# Autodesk Inventor assembly: FrontOdomPod
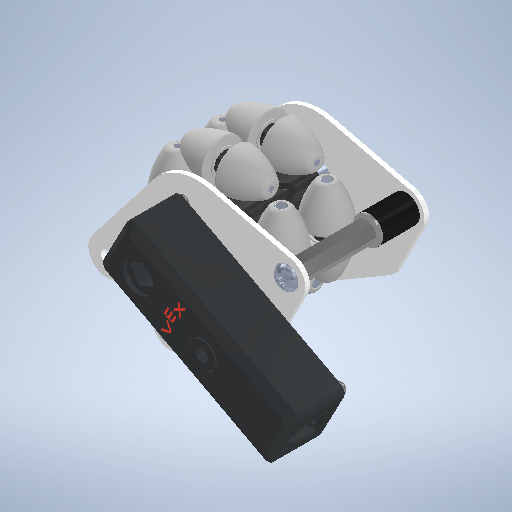
[picture p0: Inventor's stored thumbnail of the model, 512x512]
Saved by Autodesk Inventor 2025.2 (Build 292293000, 293)
## iProperties
Created: 2025-03-23
Part Number: FrontOdomPod
Document SubType Name: Assembly
Designer: roejo
Author: roejo
## Documents named in this file (18)
- C:\1629X-7700R-Worlds-Bot\Bot 1\FrontOdomPod.iam
- C:\1629X-7700R-Worlds-Bot\Bot 1\Plastic\Odom\Front Horizontal Odom Pod nonRot Side.ipt
- C:\1629X-7700R-Worlds-Bot\Bot 1\Plastic\Odom\Front Horizontal Odom Pod Rot Side.ipt
- C:\1629X-7700R-Worlds-Bot\VEX-CAD-Inventor-1.4.2\Motion\Spacers\Washer Steel\SWasher .375 OD x .031250.ipt
- C:\1629X-7700R-Worlds-Bot\VEX-CAD-Inventor-1.4.2\Motion\Spacers\Washer Steel.ipt
- C:\1629X-7700R-Worlds-Bot\VEX-CAD-Inventor-1.4.2\Structure\Standoff\Standoff 1.00.ipt
- C:\1629X-7700R-Worlds-Bot\VEX-CAD-Inventor-1.4.2\Structure\Standoff.ipt
- C:\1629X-7700R-Worlds-Bot\VEX-CAD-Inventor-1.4.2\Motion\Spacers\Spacer Nylon .375 OD\NSpacer .375 OD x .500.ipt
- C:\1629X-7700R-Worlds-Bot\VEX-CAD-Inventor-1.4.2\Motion\Spacers\Spacer Nylon .375 OD.ipt
- C:\1629X-7700R-Worlds-Bot\VEX-CAD-Inventor-1.4.2\Electronics\Sensors\V5 Rotation Sensor.ipt
- C:\1629X-7700R-Worlds-Bot\VEX-CAD-Inventor-1.4.2\Motion\Wheels\Omni Wheel\2 Omni AS, No Insert.ipt
- C:\1629X-7700R-Worlds-Bot\VEX-CAD-Inventor-1.4.2\Motion\Shaft LS\Shaft Collar Metal\Shaft Collar No Screw.iam
- C:\1629X-7700R-Worlds-Bot\VEX-CAD-Inventor-1.4.2\Motion\Shaft LS\Shaft Collar Metal.iam
- C:\1629X-7700R-Worlds-Bot\VEX-CAD-Inventor-1.4.2\Motion\Spacers\Washer Teflon\TWasher .375 OD x .04000.ipt
- C:\1629X-7700R-Worlds-Bot\VEX-CAD-Inventor-1.4.2\Motion\Spacers\Washer Teflon.ipt
- C:\1629X-7700R-Worlds-Bot\VEX-CAD-Inventor-1.4.2\Structure\Hardware\Screw Steel - Star.ipt
- C:\1629X-7700R-Worlds-Bot\VEX-CAD-Inventor-1.4.2\Structure\Hardware\Screw Steel - Star\SScrew Star Smooth .375.ipt
- C:\1629X-7700R-Worlds-Bot\VEX-CAD-Inventor-1.4.2\Structure\Hardware\Screw Steel - Star\SScrew Star Smooth .875.ipt
## Components (19 placed, 11 different names)
1. Front Horizontal Odom Pod nonRot Side:1 — Insert:5, Insert:11, Insert:12, Insert:17, Insert:18
2. Front Horizontal Odom Pod Rot Side:1 — Insert:1, Insert:9, Insert:10, Insert:19, Insert:20
3. SWasher .375 OD x .031250:1 — Insert:3, Insert:4
4. SWasher .375 OD x .031250:2 — Insert:1, Insert:2
5. Standoff 1.00:1 — Insert:2, Insert:3
6. NSpacer .375 OD x .500:1 — Insert:4, Insert:5
7. SWasher .375 OD x .031250:3
8. SWasher .375 OD x .031250:4 — Insert:9
9. Standoff 1.00:2
10. NSpacer .375 OD x .500:2 — Insert:11
11. V5 Rotation Sensor:1 — Insert:10
12. 2 Omni AS, No Insert:1 — Insert:13, Insert:14
13. Shaft Collar No Screw:1 [sub-assembly] — Insert:12, Insert:13
14. 2 Omni AS, No Insert:2 — Insert:14, Insert:15
15. TWasher .375 OD x .04000:1 — Insert:15
16. SScrew Star Smooth .375:3 — Insert:19
17. SScrew Star Smooth .375:4 — Insert:20
18. SScrew Star Smooth .875:6 — Insert:18
19. SScrew Star Smooth .875:7 — Insert:17
## Relationships (19: Insert 19)
- Insert:1: Front Horizontal Odom Pod Rot Side:1 ↔ SWasher .375 OD x .031250:2
- Insert:2: SWasher .375 OD x .031250:2 ↔ Standoff 1.00:1
- Insert:3: SWasher .375 OD x .031250:1 ↔ Standoff 1.00:1
- Insert:4: SWasher .375 OD x .031250:1 ↔ NSpacer .375 OD x .500:1
- Insert:5: Front Horizontal Odom Pod nonRot Side:1 ↔ NSpacer .375 OD x .500:1
- [Insert]: SWasher .375 OD x .031250:4 ↔ Standoff 1.00:2
- [Insert]: SWasher .375 OD x .031250:3 ↔ Standoff 1.00:2
- [Insert]: SWasher .375 OD x .031250:3 ↔ NSpacer .375 OD x .500:2
- Insert:9: Front Horizontal Odom Pod Rot Side:1 ↔ SWasher .375 OD x .031250:4
- Insert:10: Front Horizontal Odom Pod Rot Side:1 ↔ V5 Rotation Sensor:1
- Insert:11: Front Horizontal Odom Pod nonRot Side:1 ↔ NSpacer .375 OD x .500:2
- Insert:12: Front Horizontal Odom Pod nonRot Side:1 ↔ Shaft Collar No Screw:1
- Insert:13: 2 Omni AS, No Insert:1 ↔ Shaft Collar No Screw:1
- Insert:14: 2 Omni AS, No Insert:1 ↔ 2 Omni AS, No Insert:2
- Insert:15: 2 Omni AS, No Insert:2 ↔ TWasher .375 OD x .04000:1
- Insert:17: Front Horizontal Odom Pod nonRot Side:1 ↔ SScrew Star Smooth .875:7
- Insert:18: Front Horizontal Odom Pod nonRot Side:1 ↔ SScrew Star Smooth .875:6
- Insert:19: Front Horizontal Odom Pod Rot Side:1 ↔ SScrew Star Smooth .375:3
- Insert:20: Front Horizontal Odom Pod Rot Side:1 ↔ SScrew Star Smooth .375:4
## Named parameters: d5_d1 = 0 mm, d6_d2 = 0 mm, d7_d3 = 0 mm
